# Autodesk Inventor assembly: Drive Assembly
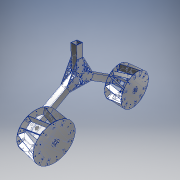
[picture p0: Inventor's stored thumbnail of the model, 180x180]
Saved by Autodesk Inventor 2019 (Build 230136000, 136)
## iProperties
Created: 2018-09-22
Part Number: Drive Assembly
Document SubType Name: Assembly
Designer: Adhik
Mass: 4735.4 g
Surface Area: 16487.1 cm^2
Volume: 1783.39 cm^3
Density: 2.65528 g/cm^3
Author: Adhik
## Documents named in this file (7)
- C:\Users\Adhik\Documents\CAD\Julie\Drive Assembly.iam
- C:\Users\Adhik\Documents\CAD\Julie\Outer Gusset Plate.ipt
- C:\Users\Adhik\Documents\CAD\Julie\Arm 18 inch.ipt
- C:\Users\Adhik\Documents\CAD\Julie\Arm 4 inch.ipt
- C:\Users\Adhik\Documents\CAD\Julie\Arm 8 inch.ipt
- C:\Users\Adhik\Documents\CAD\Julie\Drive Bearing.ipt
- C:\Users\Adhik\Documents\CAD\Julie\Wheel.iam
## Components (13 placed, 6 different names)
1. Outer Gusset Plate:1 — Mate:1, Mate:3, Mate:9, Mate:10, Mate:11, Mate:12, Mate:14, Mate:15, Mate:19
2. Arm 18 inch:1 — Mate:1, Mate:3, Mate:7, Mate:19
3. Arm 4 inch:1 — Mate:7, Insert:3, Insert:4
4. Arm 4 inch:2 — Mate:13, Flush:3, Flush:4, Insert:1, Insert:2
5. Arm 8 inch:1 — Mate:9, Mate:10, Mate:11, Mate:16, Mate:17, Mate:18
6. Arm 18 inch:2 — Mate:12, Mate:13, Flush:3, Flush:4, Mate:14, Mate:15
7. Outer Gusset Plate:2 — Mate:16, Mate:17, Mate:18
8. Drive Bearing:1 — Insert:1, Mate:20
9. Drive Bearing:2 — Insert:2
10. Drive Bearing:3 — Insert:4
11. Drive Bearing:4 — Insert:3, Mate:21
12. Wheel:1 [sub-assembly] — Mate:21, Flush:5
13. Wheel:2 [sub-assembly] — Mate:20, Flush:5
## Relationships (23: Mate 16, Insert 4, Flush 3)
- Mate:1: Outer Gusset Plate:1 ↔ Arm 18 inch:1
- Mate:3: Outer Gusset Plate:1 ↔ Arm 18 inch:1
- Mate:7: Arm 18 inch:1 ↔ Arm 4 inch:1
- Mate:9: Outer Gusset Plate:1 ↔ Arm 8 inch:1
- Mate:10: Outer Gusset Plate:1 ↔ Arm 8 inch:1
- Mate:11: Outer Gusset Plate:1 ↔ Arm 8 inch:1
- Mate:12: Outer Gusset Plate:1 ↔ Arm 18 inch:2
- Mate:13: Arm 4 inch:2 ↔ Arm 18 inch:2
- Flush:3: Arm 4 inch:2 ↔ Arm 18 inch:2
- Flush:4: Arm 4 inch:2 ↔ Arm 18 inch:2
- Mate:14: Outer Gusset Plate:1 ↔ Arm 18 inch:2
- Mate:15: Outer Gusset Plate:1 ↔ Arm 18 inch:2
- Mate:16: Arm 8 inch:1 ↔ Outer Gusset Plate:2
- Mate:17: Arm 8 inch:1 ↔ Outer Gusset Plate:2
- Mate:18: Arm 8 inch:1 ↔ Outer Gusset Plate:2
- Mate:19: Outer Gusset Plate:1 ↔ Arm 18 inch:1
- Insert:1: Arm 4 inch:2 ↔ Drive Bearing:1
- Insert:2: Arm 4 inch:2 ↔ Drive Bearing:2
- Insert:3: Arm 4 inch:1 ↔ Drive Bearing:4
- Insert:4: Arm 4 inch:1 ↔ Drive Bearing:3
- Mate:20: Drive Bearing:1 ↔ Wheel:2
- Mate:21: Drive Bearing:4 ↔ Wheel:1
- Flush:5: Wheel:1 ↔ Wheel:2
